# Autodesk Inventor assembly: Torre Inferior+Motor+Eix
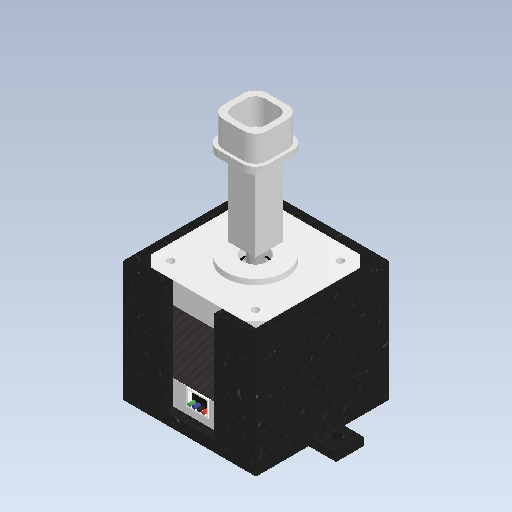
[picture p0: Inventor's stored thumbnail of the model, 512x512]
Saved by Autodesk Inventor 2021 (Build 250183000, 183)
## iProperties
Created: 2021-06-02
Part Number: Torre Inferior+Motor+Eix
Document SubType Name: Assembly
Designer: Marc
Author: Marc
## Documents named in this file (4)
- C:\Users\Marc\Documents\Projectes\Rubik's Cube Solver\Prototip Definitiu\Torre Inferior+Motor+Eix.iam
- C:\Users\Marc\Documents\Projectes\Rubik's Cube Solver\Prototip Definitiu\Components\Caixa Motor Definitiva.ipt
- C:\Users\Marc\Documents\Projectes\Rubik's Cube Solver\Prototip Definitiu\Components\Nema17\Steppermotor 17HS4417 1.7A 1.8° 2.55V v6_TOP.iam
- C:\Users\Marc\Documents\Projectes\Rubik's Cube Solver\Prototip Definitiu\Components\Eix Superior i Inferior.ipt
## Components (3 placed, 3 different names)
1. Caixa Motor Definitiva:1 — Coincidencia:1, Coincidencia:2, Coincidencia:3
2. Steppermotor 17HS4417 1.7A 1.8° 2.55V v6_TOP:1 [sub-assembly] — Coincidencia:1, Coincidencia:2, Coincidencia:3, Coincidencia:4, Coincidencia:5, Coincidencia:6
3. Eix Superior i Inferior:1 — Coincidencia:4, Coincidencia:5, Coincidencia:6
## Relationships (6: Mate 6)
- Coincidencia:1 [Mate]: Caixa Motor Definitiva:1 ↔ Steppermotor 17HS4417 1.7A 1.8° 2.55V v6_TOP:1
- Coincidencia:2 [Mate]: Caixa Motor Definitiva:1 ↔ Steppermotor 17HS4417 1.7A 1.8° 2.55V v6_TOP:1
- Coincidencia:3 [Mate]: Caixa Motor Definitiva:1 ↔ Steppermotor 17HS4417 1.7A 1.8° 2.55V v6_TOP:1
- Coincidencia:4 [Mate]: Steppermotor 17HS4417 1.7A 1.8° 2.55V v6_TOP:1 ↔ Eix Superior i Inferior:1
- Coincidencia:5 [Mate]: Steppermotor 17HS4417 1.7A 1.8° 2.55V v6_TOP:1 ↔ Eix Superior i Inferior:1
- Coincidencia:6 [Mate]: Steppermotor 17HS4417 1.7A 1.8° 2.55V v6_TOP:1 ↔ Eix Superior i Inferior:1
